# Autodesk Inventor assembly: Exhaust Filter-Unit
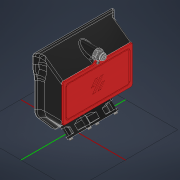
[picture p0: Inventor's stored thumbnail of the model, 180x180]
Saved by Autodesk Inventor 2022.2 (Build 262287010, 287A)
## iProperties
Created: 2022-03-16
Part Number: Exhaust Filter-Unit
Document SubType Name: Assembly
Designer: sleib
Author: sleib
## Documents named in this file (8)
- C:\Users\sleib\Projekte\Voron-2\CAD\Inventor\Exhaust Filter-Unit.iam
- C:\Users\sleib\Projekte\Voron-2\CAD\Inventor\Exhaust Housing.ipt
- C:\Users\sleib\Projekte\Voron-2\CAD\Inventor\Exhaust Cover.ipt
- C:\Users\sleib\Projekte\Voron-2\CAD\Inventor\M3 Threaded Insert.ipt
- C:\Users\sleib\Projekte\Voron-2\CAD\Inventor\M3x8 BHCS.ipt
- C:\Users\sleib\Projekte\Voron-2\CAD\Inventor\Fan 6020.iam
- C:\Users\sleib\Projekte\Voron-2\CAD\Inventor\M3x25 SHCS.ipt
- C:\Users\sleib\Projekte\Voron-2\CAD\Inventor\Bowden Connector.ipt
## Components (18 placed, 7 different names)
1. Exhaust Housing:1 — Passend:1, Passend:2, Passend:3, Passend:4, Passend:5, Winkel:1, Passend:6, Fluchtend:1, Passend:7, Passend:8, Passend:9, Passend:10, Fluchtend:2, Fluchtend:3, Fluchtend:4, Fluchtend:5, Passend:11, Passend:12, Passend:13, Passend:14, Fluchtend:6, Fluchtend:7, Fluchtend:8, Fluchtend:9, Passend:21, Passend:30, Passend:31
2. Exhaust Cover:1 — Passend:4, Passend:5, Winkel:1, Passend:16
3. M3 Threaded Insert:1 — Passend:6, Fluchtend:1, Passend:15
4. M3 Threaded Insert:2 — Passend:7, Fluchtend:5
5. M3 Threaded Insert:3 — Passend:8, Fluchtend:4
6. M3 Threaded Insert:4 — Passend:9, Fluchtend:3
7. M3 Threaded Insert:5 — Passend:10, Fluchtend:2
8. M3 Threaded Insert:6 — Passend:11, Fluchtend:8, Passend:17, Passend:25
9. M3 Threaded Insert:7 — Passend:12, Fluchtend:9, Passend:18, Passend:24
10. M3 Threaded Insert:8 — Passend:13, Fluchtend:7, Passend:19, Passend:23
11. M3 Threaded Insert:9 — Passend:14, Fluchtend:6, Passend:20, Passend:22
12. M3x8 BHCS:1 — Passend:15, Passend:16
13. Fan 6020:1 [sub-assembly] — Passend:17, Passend:18, Passend:19, Passend:20, Passend:21, Passend:26, Passend:27, Passend:28, Passend:29
14. M3x25 SHCS:1 — Passend:25, Passend:26
15. M3x25 SHCS:2 — Passend:24, Passend:27
16. M3x25 SHCS:3 — Passend:23, Passend:28
17. M3x25 SHCS:4 — Passend:22, Passend:29
18. Bowden Connector:1 — Passend:30, Passend:31
## Relationships (41: Mate 31, Flush 9, Angle 1)
- Passend:1 [Mate]: Exhaust Housing:1
- Passend:2 [Mate]: Exhaust Housing:1
- Passend:3 [Mate]: Exhaust Housing:1
- Passend:4 [Mate]: Exhaust Housing:1 ↔ Exhaust Cover:1
- Passend:5 [Mate]: Exhaust Housing:1 ↔ Exhaust Cover:1
- Winkel:1 [Angle] (0 deg): Exhaust Housing:1 ↔ Exhaust Cover:1
- Passend:6 [Mate]: Exhaust Housing:1 ↔ M3 Threaded Insert:1
- Fluchtend:1 [Flush]: Exhaust Housing:1 ↔ M3 Threaded Insert:1
- Passend:7 [Mate]: Exhaust Housing:1 ↔ M3 Threaded Insert:2
- Passend:8 [Mate]: Exhaust Housing:1 ↔ M3 Threaded Insert:3
- Passend:9 [Mate]: Exhaust Housing:1 ↔ M3 Threaded Insert:4
- Passend:10 [Mate]: Exhaust Housing:1 ↔ M3 Threaded Insert:5
- Fluchtend:2 [Flush]: Exhaust Housing:1 ↔ M3 Threaded Insert:5
- Fluchtend:3 [Flush]: Exhaust Housing:1 ↔ M3 Threaded Insert:4
- Fluchtend:4 [Flush]: Exhaust Housing:1 ↔ M3 Threaded Insert:3
- Fluchtend:5 [Flush]: Exhaust Housing:1 ↔ M3 Threaded Insert:2
- Passend:11 [Mate]: Exhaust Housing:1 ↔ M3 Threaded Insert:6
- Passend:12 [Mate]: Exhaust Housing:1 ↔ M3 Threaded Insert:7
- Passend:13 [Mate]: Exhaust Housing:1 ↔ M3 Threaded Insert:8
- Passend:14 [Mate]: Exhaust Housing:1 ↔ M3 Threaded Insert:9
- Fluchtend:6 [Flush]: Exhaust Housing:1 ↔ M3 Threaded Insert:9
- Fluchtend:7 [Flush]: Exhaust Housing:1 ↔ M3 Threaded Insert:8
- Fluchtend:8 [Flush]: Exhaust Housing:1 ↔ M3 Threaded Insert:6
- Fluchtend:9 [Flush]: Exhaust Housing:1 ↔ M3 Threaded Insert:7
- Passend:15 [Mate]: M3 Threaded Insert:1 ↔ M3x8 BHCS:1
- Passend:16 [Mate]: Exhaust Cover:1 ↔ M3x8 BHCS:1
- Passend:17 [Mate]: M3 Threaded Insert:6 ↔ Fan 6020:1
- Passend:18 [Mate]: M3 Threaded Insert:7 ↔ Fan 6020:1
- Passend:19 [Mate]: M3 Threaded Insert:8 ↔ Fan 6020:1
- Passend:20 [Mate]: M3 Threaded Insert:9 ↔ Fan 6020:1
- Passend:21 [Mate]: Exhaust Housing:1 ↔ Fan 6020:1
- Passend:22 [Mate]: M3 Threaded Insert:9 ↔ M3x25 SHCS:4
- Passend:23 [Mate]: M3 Threaded Insert:8 ↔ M3x25 SHCS:3
- Passend:24 [Mate]: M3 Threaded Insert:7 ↔ M3x25 SHCS:2
- Passend:25 [Mate]: M3 Threaded Insert:6 ↔ M3x25 SHCS:1
- Passend:26 [Mate]: Fan 6020:1 ↔ M3x25 SHCS:1
- Passend:27 [Mate]: Fan 6020:1 ↔ M3x25 SHCS:2
- Passend:28 [Mate]: Fan 6020:1 ↔ M3x25 SHCS:3
- Passend:29 [Mate]: Fan 6020:1 ↔ M3x25 SHCS:4
- Passend:30 [Mate]: Exhaust Housing:1 ↔ Bowden Connector:1
- Passend:31 [Mate]: Exhaust Housing:1 ↔ Bowden Connector:1
